# Autodesk Inventor assembly: 铲屎机
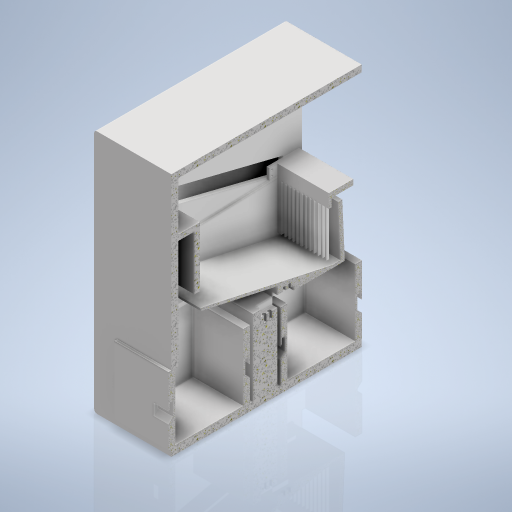
[picture p0: Inventor's stored thumbnail of the model, 512x512]
Saved by Autodesk Inventor 2023.1 (Build 271208000, 208)
## iProperties
Created: 2023-07-19
Part Number: 铲屎机
Document SubType Name: Assembly
Designer: Selcon
Author: Selcon
## Documents named in this file (8)
- C:\Users\Selcon\Desktop\hisi\铲屎机3D模型\铲屎机.iam
- C:\Users\Selcon\Desktop\hisi\铲屎机3D模型\外壳.ipt
- C:\Users\Selcon\Desktop\hisi\铲屎机3D模型\容器.ipt
- C:\Users\Selcon\Desktop\hisi\铲屎机3D模型\猫砂盆底座.ipt
- C:\Users\Selcon\Desktop\hisi\铲屎机3D模型\猫砂盆.ipt
- C:\Users\Selcon\Desktop\hisi\铲屎机3D模型\挡板.ipt
- C:\Users\Selcon\Desktop\hisi\铲屎机3D模型\猫铲.ipt
- C:\Users\Selcon\Desktop\hisi\铲屎机3D模型\外壳挡板.ipt
## Components (8 placed, 7 different names)
1. 外壳:1 — 配合:1, 配合:2, 配合:3, 配合:4, 配合:5, 配合:6, 配合:7, 配合:10, 配合:11, 配合:12, 配合:14, 表面齐平:1, 表面齐平:2
2. 容器:1 — 配合:4, 配合:5
3. 容器:2 — 配合:6, 配合:7
4. 猫砂盆底座:1 — 配合:10, 配合:11, 配合:12, 配合:13
5. 猫砂盆:1 — 配合:13, 配合:14, 旋转:1, 配合:15
6. 挡板:1 — 旋转:1
7. 猫铲:1 — 配合:15
8. 外壳挡板:1 — 表面齐平:1, 表面齐平:2
## Relationships (16: Mate 13, Flush 2, RevoluteJoint 1)
- 配合:1 [Mate]: 外壳:1
- 配合:2 [Mate]: 外壳:1
- 配合:3 [Mate]: 外壳:1
- 配合:4 [Mate]: 外壳:1 ↔ 容器:1
- 配合:5 [Mate]: 外壳:1 ↔ 容器:1
- 配合:6 [Mate]: 外壳:1 ↔ 容器:2
- 配合:7 [Mate]: 外壳:1 ↔ 容器:2
- 配合:10 [Mate]: 外壳:1 ↔ 猫砂盆底座:1
- 配合:11 [Mate]: 外壳:1 ↔ 猫砂盆底座:1
- 配合:12 [Mate]: 外壳:1 ↔ 猫砂盆底座:1
- 配合:13 [Mate]: 猫砂盆底座:1 ↔ 猫砂盆:1
- 配合:14 [Mate]: 外壳:1 ↔ 猫砂盆:1
- 旋转:1 [RevoluteJoint]: 猫砂盆:1 ↔ 挡板:1
- 配合:15 [Mate]: 猫砂盆:1 ↔ 猫铲:1
- 表面齐平:1 [Flush]: 外壳:1 ↔ 外壳挡板:1
- 表面齐平:2 [Flush]: 外壳:1 ↔ 外壳挡板:1
